# Autodesk Inventor assembly: Full
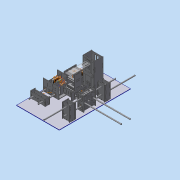
[picture p0: Inventor's stored thumbnail of the model, 180x180]
Saved by Autodesk Inventor 2016 SP1 (Build 200210100, 210)
## iProperties
Created: 2016-02-23
Part Number: Full
Document SubType Name: Assembly
Designer: Mohamed A.
Author: Mohamed A.
## Documents named in this file (14)
- C:\Users\Mohamed\Documents\inventor\Faboscope\Full.iam
- C:\Users\Mohamed\Documents\inventor\Faboscope\Laser Cut\Floor.ipt
- C:\Users\Mohamed\Documents\inventor\Faboscope\Laser Cut\X-Motor-Housing\X-Motor-Housing.iam
- C:\Users\Mohamed\Documents\inventor\Faboscope\Laser Cut\Y-Motor-Housing\new\Y-Motor-Housing.iam
- C:\Users\Mohamed\Documents\inventor\Faboscope\Laser Cut\X-Anchor\Mirrored\X-Anchor.iam
- C:\Users\Mohamed\Documents\inventor\Faboscope\Laser Cut\Camera-Holder\Camera-Holder.iam
- C:\Users\Mohamed\Documents\inventor\Faboscope\Laser Cut\Y-Shafts-Holder\Y-Shafts-Holder.iam
- C:\Users\Mohamed\Documents\inventor\StemCellsPlatform\Shafts\Shaft.ipt
- C:\Users\Mohamed\Documents\inventor\Faboscope\Shafts\Shaft-081.ipt
- C:\Users\Mohamed\Documents\inventor\Faboscope\Laser Cut\Y-Anchor\Y-Anchor.iam
- C:\Users\Mohamed\Documents\inventor\Faboscope\Shafts\Shaft-083.ipt
- C:\Users\Mohamed\Documents\inventor\Faboscope\Shafts\Shaft-084.ipt
- C:\Users\Mohamed\Documents\inventor\Faboscope\Shafts\Shaft-085.ipt
- C:\Users\Mohamed\Documents\inventor\Faboscope\Laser Cut\Slider Holder\Slider-Holder.iam
## Components (15 placed, 12 different names)
1. Floor:1 — Flush:3, Flush:4, Flush:7, Flush:9, Angle:1, Flush:16, Mate:31, Flush:17, Flush:27, Flush:28
2. X-Motor-Housing:1 [sub-assembly] — Flush:3, Flush:4, Mate:15, Mate:17, Angle:1, Flush:10, Flush:11, Mate:29, Symmetry:1, Mate:34, Mate:35, Flush:17, Flush:18
3. Y-Motor-Housing:1 [sub-assembly] — X-Axis, Cylindrical:8, Mate:19, Mate:20, Flush:12, Flush:13, Mate:30
4. X-Anchor:1 [sub-assembly] — Mate:16, Mate:18, Mate:29, Symmetry:1, Mate:35, Flush:19
5. Camera-Holder:1 [sub-assembly] — Cylindrical:9, Y-Axis, Mate:27, Mate:28, Flush:20, Flush:21, Flush:22, Flush:23, Flush:25, Mate:36, Mate:37
6. Y-Shafts-Holder:1 [sub-assembly] — Mate:25, Mate:26, Mate:28, Mate:32, Flush:19
7. Y-Shafts-Holder:2 [sub-assembly] — Flush:7, Flush:9, Mate:13, Mate:14, Flush:16, Mate:27, Mate:33, Mate:34, Flush:18
8. Shaft-081:1 — Mate:13, Cylindrical:11, Mate:25
9. Shaft-081:2 — Mate:14, Cylindrical:12, Mate:26
10. Shaft-084:3 — Mate:17, Mate:18, Flush:11, Cylindrical:8
11. Shaft-085:4 — Mate:15, Mate:16, Flush:10, X-Axis
12. Shaft-083:5 — Mate:19, Cylindrical:9, Flush:12, Mate:22
13. Shaft-083:6 — Mate:20, Y-Axis, Flush:13, Mate:21
14. Y-Anchor:1 [sub-assembly] — Mate:21, Mate:22, Cylindrical:11, Cylindrical:12, Mate:30, Mate:32, Mate:33
15. Slider-Holder:1 [sub-assembly] — Flush:26, Mate:37, Mate:38, Flush:27, Flush:28
## Relationships (54: Mate 24, Flush 20, CylindricalJoint 6, Symmetry 3, Angle 1)
- Flush:3: Floor:1 ↔ X-Motor-Housing:1
- Flush:4: Floor:1 ↔ X-Motor-Housing:1
- Flush:7: Floor:1 ↔ Y-Shafts-Holder:2
- Flush:9 (30 mm): Floor:1 ↔ Y-Shafts-Holder:2
- Mate:13: Y-Shafts-Holder:2 ↔ Shaft-081:1
- Mate:14: Y-Shafts-Holder:2 ↔ Shaft-081:2
- Mate:15: X-Motor-Housing:1 ↔ Shaft-085:4
- Mate:16: X-Anchor:1 ↔ Shaft-085:4
- Mate:17: X-Motor-Housing:1 ↔ Shaft-084:3
- Mate:18: X-Anchor:1 ↔ Shaft-084:3
- Angle:1 (0 deg): Floor:1 ↔ X-Motor-Housing:1
- Flush:10: X-Motor-Housing:1 ↔ Shaft-085:4
- Flush:11: X-Motor-Housing:1 ↔ Shaft-084:3
- X-Axis [CylindricalJoint]: Y-Motor-Housing:1 ↔ Shaft-085:4
- Cylindrical:8: Y-Motor-Housing:1 ↔ Shaft-084:3
- Mate:19: Y-Motor-Housing:1 ↔ Shaft-083:5
- Mate:20: Y-Motor-Housing:1 ↔ Shaft-083:6
- Cylindrical:9: Camera-Holder:1 ↔ Shaft-083:5
- Y-Axis [CylindricalJoint]: Camera-Holder:1 ↔ Shaft-083:6
- Flush:12: Y-Motor-Housing:1 ↔ Shaft-083:5
- Flush:13: Y-Motor-Housing:1 ↔ Shaft-083:6
- Flush:16 (15 mm): Floor:1 ↔ Y-Shafts-Holder:2
- Mate:21: Shaft-083:6 ↔ Y-Anchor:1
- Mate:22: Shaft-083:5 ↔ Y-Anchor:1
- Cylindrical:11: Shaft-081:1 ↔ Y-Anchor:1
- Cylindrical:12: Shaft-081:2 ↔ Y-Anchor:1
- Mate:25: Y-Shafts-Holder:1 ↔ Shaft-081:1
- Mate:26: Y-Shafts-Holder:1 ↔ Shaft-081:2
- Mate:27 (7 mm): Camera-Holder:1 ↔ Y-Shafts-Holder:2
- Mate:28 (7 mm): Camera-Holder:1 ↔ Y-Shafts-Holder:1
- Mate:29 (195 mm): X-Motor-Housing:1 ↔ X-Anchor:1
- Mate:30 (155 mm): Y-Motor-Housing:1 ↔ Y-Anchor:1
- Symmetry:1: X-Motor-Housing:1 ↔ X-Anchor:1
- Mate:31: Floor:1
- Mate:32 (5 mm): Y-Shafts-Holder:1 ↔ Y-Anchor:1
- Mate:33 (5 mm): Y-Shafts-Holder:2 ↔ Y-Anchor:1
- Mate:34 (-285 mm): X-Motor-Housing:1 ↔ Y-Shafts-Holder:2
- Mate:35 (-320 mm): X-Motor-Housing:1 ↔ X-Anchor:1
- Flush:17 (7.5 mm): Floor:1 ↔ X-Motor-Housing:1
- Flush:18: X-Motor-Housing:1 ↔ Y-Shafts-Holder:2
- Flush:19: X-Anchor:1 ↔ Y-Shafts-Holder:1
- Flush:20: Camera-Holder:1
- Flush:21: Camera-Holder:1
- Flush:22: Camera-Holder:1
- Flush:23: Camera-Holder:1
- Symmetry:2
- Symmetry:3
- Flush:25: Camera-Holder:1
- Mate:36: Camera-Holder:1
- Flush:26: Slider-Holder:1
- Mate:37: Camera-Holder:1 ↔ Slider-Holder:1
- Mate:38: Slider-Holder:1
- Flush:27: Floor:1 ↔ Slider-Holder:1
- Flush:28: Floor:1 ↔ Slider-Holder:1
